# Autodesk Inventor assembly: A2017_T2_06
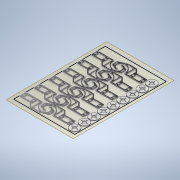
[picture p0: Inventor's stored thumbnail of the model, 180x180]
Saved by Autodesk Inventor 2022.3 (Build 263350000, 350)
## iProperties
Created: 2022-09-28
Part Number: A2017_T2_06
Document SubType Name: Assembly
Designer: Masato
Author: Masato
## Documents named in this file (4)
- C:\Users\Masato\Documents\Inventor\Inventor for CIT Brains\SUSTAINA-OP - cam\Cam\A2017_T2\A2017_T2_06.iam
- C:\Users\Masato\Documents\Inventor\Inventor for CIT Brains\SUSTAINA-OP - cam\Cam\DisposableBoard.ipt
- C:\Users\Masato\Documents\Inventor\Inventor for CIT Brains\SUSTAINA-OP - cam\LowerBody\Ankle\Ankle_side_frame.ipt
- C:\Users\Masato\Documents\Inventor\Inventor for CIT Brains\SUSTAINA-OP - cam\UpperBody\Trunk\CrossRollerBearing\Inner_flange.ipt
## Components (22 placed, 3 different names)
1. DisposableBoard:1 — フラッシュ:1, フラッシュ:2, フラッシュ:3, フラッシュ:4, フラッシュ:5, フラッシュ:6, 正接:3
2. Inner_flange:1 — メイト:4, 正接:1, 正接:2, 角度:1, 正接:3
3. Inner_flange:2
4. Inner_flange:3
5. Inner_flange:4
6. Inner_flange:5
7. Inner_flange:6
8. Inner_flange:7
9. Inner_flange:8
10. Inner_flange:9
11. Ankle_side_frame:2 — メイト:1, 正接:1, 角度:2, 正接:4
12. Ankle_side_frame:13 — フラッシュ:5, メイト:5, フラッシュ:6, 正接:2, 角度:2, 正接:4
13. Ankle_side_frame:14
14. Ankle_side_frame:15
15. Ankle_side_frame:16
16. Ankle_side_frame:17
17. Ankle_side_frame:18
18. Ankle_side_frame:19
19. Ankle_side_frame:20
20. Ankle_side_frame:21
21. Ankle_side_frame:22
22. Ankle_side_frame:23
## Component patterns: (9 elements, first: Inner_flange:1), (6 elements, first: Ankle_side_frame:2 + Ankle_side_frame:13)
## Relationships (15: Flush 6, Tangent 4, Mate 3, Angle 2)
- フラッシュ:1 [Flush]: DisposableBoard:1
- フラッシュ:2 [Flush]: DisposableBoard:1
- フラッシュ:3 [Flush]: DisposableBoard:1
- フラッシュ:4 [Flush]: DisposableBoard:1
- メイト:1 [Mate]: Ankle_side_frame:2
- フラッシュ:5 [Flush] (-2 mm): DisposableBoard:1 ↔ Ankle_side_frame:13
- フラッシュ:6 [Flush] (-2 mm): DisposableBoard:1 ↔ Ankle_side_frame:13
- メイト:4 [Mate]: Inner_flange:1
- メイト:5 [Mate]: Ankle_side_frame:13
- 正接:1 [Tangent] (2.1 mm): Inner_flange:1 ↔ Ankle_side_frame:2
- 正接:2 [Tangent]: Inner_flange:1 ↔ Ankle_side_frame:13
- 角度:1 [Angle] (0 deg): Inner_flange:1
- 角度:2 [Angle] (0 deg): Ankle_side_frame:2 ↔ Ankle_side_frame:13
- 正接:3 [Tangent] (2 mm): DisposableBoard:1 ↔ Inner_flange:1
- 正接:4 [Tangent] (2.1 mm): Ankle_side_frame:2 ↔ Ankle_side_frame:13
